# Autodesk Inventor assembly: centralLineAssy
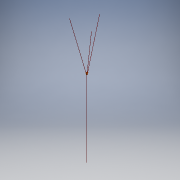
[picture p0: Inventor's stored thumbnail of the model, 180x180]
Saved by Autodesk Inventor 2016 (Build 200138000, 138)
## iProperties
Created: 2015-10-15
Part Number: centralLineAssy
Document SubType Name: Assembly
Designer: ddeboer
Author: ddeboer
## Documents named in this file (4)
- C:\Users\krosie\Google Drive\HERA\hera-cad\feed\centralLineAssy.iam
- C:\Users\krosie\Google Drive\HERA\hera-cad\feed\centralLineLower.ipt
- C:\Users\krosie\Google Drive\HERA\hera-cad\feed\centralLineSplitter.ipt
- C:\Users\krosie\Google Drive\HERA\hera-cad\feed\centralLineUpper.ipt
## Components (5 placed, 3 different names)
1. centralLineLower:1 — Insert:1
2. centralLineSplitter:1 — Insert:1, Mate:1
3. centralLineUpper:1 — Mate:1
4. centralLineUpper:2
5. centralLineUpper:3
## Component patterns: (3 elements, first: centralLineUpper:1)
## Relationships (2: Insert 1, Mate 1)
- Insert:1 (-10 mm): centralLineLower:1 ↔ centralLineSplitter:1
- Mate:1: centralLineSplitter:1 ↔ centralLineUpper:1
